# Autodesk Inventor assembly: MK3-Swerve-Module-Falcons-&-Neos
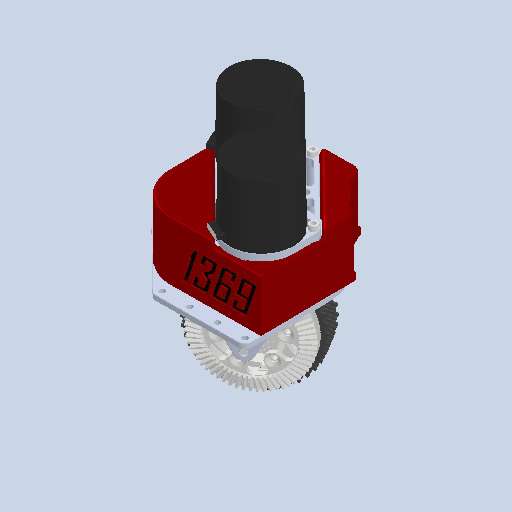
[picture p0: Inventor's stored thumbnail of the model, 512x512]
Saved by Autodesk Inventor 2024 (Build 280153000, 153)
## iProperties
Created: 2024-01-06
Part Number: MK3-Swerve-Module-Falcons-&-Neos
Document SubType Name: Assembly
Designer: rohan
Author: rohan
## Documents named in this file (27)
- C:\Users\5652160\OneDrive - Hillsborough County Public Schools\Robotics\FIRST-Robotics-Competition\Crescendo\Minotaur-Crescendo-Robot\Motion\Swerve-Modules\MK3-Swerve-Module-Neos.iam
- C:\Users\5652160\OneDrive - Hillsborough County Public Schools\Robotics\FIRST-Robotics-Competition\Crescendo\Minotaur-Crescendo-Robot\Motion\Swerve-Modules\SDS MK3 Swerve Module, Falcons, HG\MK3 Plates(Both Plates With Chamfers.ipt
- C:\Users\5652160\OneDrive - Hillsborough County Public Schools\Robotics\FIRST-Robotics-Competition\Crescendo\Minotaur-Crescendo-Robot\Electronics\NEO-Brushless-Motor.ipt
- C:\Users\5652160\OneDrive - Hillsborough County Public Schools\Robotics\FIRST-Robotics-Competition\Crescendo\Minotaur-Crescendo-Robot\Motion\Swerve-Modules\SDS MK3 Swerve Module, Falcons, HG\Spacer, #10 X 1.875, .3125 OD, 92510.ipt
- C:\Users\5652160\OneDrive - Hillsborough County Public Schools\Robotics\FIRST-Robotics-Competition\Crescendo\Minotaur-Crescendo-Robot\Motion\Swerve-Modules\SDS MK3 Swerve Module, Falcons, HG\Screw, 10-32 X 2.5, 91251A355-1.ipt
- C:\Users\5652160\OneDrive - Hillsborough County Public Schools\Robotics\FIRST-Robotics-Competition\Crescendo\Minotaur-Crescendo-Robot\Motion\Swerve-Modules\SDS MK3 Swerve Module, Falcons, HG\Screw, 10-32 X .375, 91251A340-1.ipt
- C:\Users\5652160\OneDrive - Hillsborough County Public Schools\Robotics\FIRST-Robotics-Competition\Crescendo\Minotaur-Crescendo-Robot\Motion\Swerve-Modules\SDS MK3 Swerve Module, Falcons, HG\Gear, 20DP, 16T, Falcon Spline, am-4.ipt
- C:\Users\5652160\OneDrive - Hillsborough County Public Schools\Robotics\FIRST-Robotics-Competition\Crescendo\Minotaur-Crescendo-Robot\Motion\Swerve-Modules\SDS MK3 Swerve Module, Falcons, HG\Double Gear, 20DP, 28T, 48T.ipt
- C:\Users\5652160\OneDrive - Hillsborough County Public Schools\Robotics\FIRST-Robotics-Competition\Crescendo\Minotaur-Crescendo-Robot\Motion\Swerve-Modules\SDS MK3 Swerve Module, Falcons, HG\Bearing, 6802-1.ipt
- C:\Users\5652160\OneDrive - Hillsborough County Public Schools\Robotics\FIRST-Robotics-Competition\Crescendo\Minotaur-Crescendo-Robot\Motion\Swerve-Modules\SDS MK3 Swerve Module, Falcons, HG\MK3 Center Column-1.ipt
- C:\Users\5652160\OneDrive - Hillsborough County Public Schools\Robotics\FIRST-Robotics-Competition\Crescendo\Minotaur-Crescendo-Robot\Motion\Swerve-Modules\SDS MK3 Swerve Module, Falcons, HG\Bearing, A035XPO_SA035XPO-1.ipt
- C:\Users\5652160\OneDrive - Hillsborough County Public Schools\Robotics\FIRST-Robotics-Competition\Crescendo\Minotaur-Crescendo-Robot\Motion\Swerve-Modules\SDS MK3 Swerve Module, Falcons, HG\MK3 Base Pulley-1.ipt
- C:\Users\5652160\OneDrive - Hillsborough County Public Schools\Robotics\FIRST-Robotics-Competition\Crescendo\Minotaur-Crescendo-Robot\Motion\Swerve-Modules\SDS MK3 Swerve Module, Falcons, HG\SDS 4in Wheel Assembly-1.iam
- C:\Users\5652160\OneDrive - Hillsborough County Public Schools\Robotics\FIRST-Robotics-Competition\Crescendo\Minotaur-Crescendo-Robot\Motion\Swerve-Modules\SDS MK3 Swerve Module, Falcons, HG\Gear, Bevel, KSB1.5-6015, VersaHub, .ipt
- C:\Users\5652160\OneDrive - Hillsborough County Public Schools\Robotics\FIRST-Robotics-Competition\Crescendo\Minotaur-Crescendo-Robot\Motion\Swerve-Modules\SDS MK3 Swerve Module, Falcons, HG\Bearing, am-0573, 217-2732-1.ipt
- C:\Users\5652160\OneDrive - Hillsborough County Public Schools\Robotics\FIRST-Robotics-Competition\Crescendo\Minotaur-Crescendo-Robot\Motion\Swerve-Modules\SDS MK3 Swerve Module, Falcons, HG\Wheel Mount A(Default)-1.ipt
- C:\Users\5652160\OneDrive - Hillsborough County Public Schools\Robotics\FIRST-Robotics-Competition\Crescendo\Minotaur-Crescendo-Robot\Motion\Swerve-Modules\SDS MK3 Swerve Module, Falcons, HG\Screw, Shoulder, .375 X 2.5, 5_16-18.ipt
- C:\Users\5652160\OneDrive - Hillsborough County Public Schools\Robotics\FIRST-Robotics-Competition\Crescendo\Minotaur-Crescendo-Robot\Motion\Swerve-Modules\SDS MK3 Swerve Module, Falcons, HG\MK1 Wheel Spacer-1.ipt
- C:\Users\5652160\OneDrive - Hillsborough County Public Schools\Robotics\FIRST-Robotics-Competition\Crescendo\Minotaur-Crescendo-Robot\Motion\Swerve-Modules\SDS MK3 Swerve Module, Falcons, HG\Bearing, FR8, am-0030, 217-3875-1.ipt
- C:\Users\5652160\OneDrive - Hillsborough County Public Schools\Robotics\FIRST-Robotics-Competition\Crescendo\Minotaur-Crescendo-Robot\Motion\Swerve-Modules\SDS MK3 Swerve Module, Falcons, HG\Wheel Mount B(Default)-1.ipt
- C:\Users\5652160\OneDrive - Hillsborough County Public Schools\Robotics\FIRST-Robotics-Competition\Crescendo\Minotaur-Crescendo-Robot\Motion\Swerve-Modules\SDS MK3 Swerve Module, Falcons, HG\Screw, .25-20 X 1 Socket, 91251A542-.ipt
- C:\Users\5652160\OneDrive - Hillsborough County Public Schools\Robotics\FIRST-Robotics-Competition\Crescendo\Minotaur-Crescendo-Robot\Motion\Swerve-Modules\SDS MK3 Swerve Module, Falcons, HG\Bearing, F689-ZZ-1.ipt
- C:\Users\5652160\OneDrive - Hillsborough County Public Schools\Robotics\FIRST-Robotics-Competition\Crescendo\Minotaur-Crescendo-Robot\Motion\Swerve-Modules\SDS MK3 Swerve Module, Falcons, HG\Gear, 32DP, 32T, .375 Hex Bore-1.ipt
- C:\Users\5652160\OneDrive - Hillsborough County Public Schools\Robotics\FIRST-Robotics-Competition\Crescendo\Minotaur-Crescendo-Robot\Motion\Swerve-Modules\SDS MK3 Swerve Module, Falcons, HG\MK2 Steering Shaft V3 Assembly-1.iam
- C:\Users\5652160\OneDrive - Hillsborough County Public Schools\Robotics\FIRST-Robotics-Competition\Crescendo\Minotaur-Crescendo-Robot\Motion\Swerve-Modules\SDS MK3 Swerve Module, Falcons, HG\Belt, 320-5M-09-1.ipt
- C:\Users\5652160\OneDrive - Hillsborough County Public Schools\Robotics\FIRST-Robotics-Competition\Crescendo\Minotaur-Crescendo-Robot\Structure\3D-Printed-Components\MK3-Swerve-Guard.ipt
- C:\Users\5652160\OneDrive - Hillsborough County Public Schools\Robotics\FIRST-Robotics-Competition\Crescendo\Minotaur-Crescendo-Robot\Electronics\CANcoder-Assembled.iam
## Components (37 placed, 26 different names)
1. MK3 Plates(Both Plates With Chamfers:1 — Mate:4, Mate:5, Mate:6, Mate:7, Mate:8, Mate:9, Mate:10, Mate:11, Mate:12, Mate:13, Mate:14, Mate:15, Mate:16, Mate:19, Mate:20, Mate:23, Mate:24, Mate:39, Mate:42, Mate:49, Mate:50, Mate:77, Mate:78, Mate:87, Mate:91, Mate:93, Mate:96, Mate:99, Mate:100
2. NEO-Brushless-Motor:1 — Mate:4, Mate:5, Mate:6, Mate:25
3. Spacer, #10 X 1.875, .3125 OD, 92510:1 — Mate:10, Mate:12, Mate:18
4. Spacer, #10 X 1.875, .3125 OD, 92510:2 — Mate:9, Mate:14, Mate:22, Mate:95
5. Spacer, #10 X 1.875, .3125 OD, 92510:3 — Mate:8, Mate:13, Mate:17
6. Spacer, #10 X 1.875, .3125 OD, 92510:4 — Mate:7, Mate:11, Mate:21, Mate:94
7. Screw, 10-32 X 2.5, 91251A355-1:1 — Mate:20, Mate:22
8. Screw, 10-32 X 2.5, 91251A355-1:2 — Mate:19, Mate:21, Mate:97
9. Screw, 10-32 X 2.5, 91251A355-1:3 — Mate:16, Mate:17
10. Screw, 10-32 X 2.5, 91251A355-1:4 — Mate:15, Mate:18
11. Screw, 10-32 X .375, 91251A340-1:1 — Mate:23, Mate:91, Mate:98
12. Screw, 10-32 X .375, 91251A340-1:2 — Mate:24, Mate:25
13. Gear, 20DP, 16T, Falcon Spline, am-4:1 — Mate:92
14. Double Gear, 20DP, 28T, 48T:1 — Mate:35, Mate:36, Mate:37, Mate:38, Mate:47, Mate:48
15. Bearing, 6802-1:1 — Mate:35, Mate:36
16. Bearing, 6802-1:2 — Mate:37, Mate:38
17. MK3 Center Column-1:1 — Mate:39, Mate:40, Mate:41, Mate:42, Mate:47, Mate:48, Mate:51, Mate:52, Mate:53, Mate:54
18. Bearing, 6802-1:3 — Mate:40, Mate:41
19. Bearing, A035XPO_SA035XPO-1:1 — Mate:49, Mate:50
20. MK3 Base Pulley-1:1 — Mate:51, Mate:52, Mate:53, Mate:54, Mate:70, Mate:71, Mate:72, Mate:84
21. SDS 4in Wheel Assembly-1:1 [sub-assembly] — Mate:55, Mate:56, Mate:57, Mate:58, Mate:59, Mate:64, Mate:65
22. Gear, Bevel, KSB1.5-6015, VersaHub, :1 — Mate:55, Mate:56, Mate:57
23. Bearing, am-0573, 217-2732-1:1 — Mate:58, Mate:59, Mate:60, Mate:61
24. Wheel Mount A(Default)-1:1 — Mate:60, Mate:61, Mate:62, Mate:63, Mate:70, Mate:73, Mate:74, Mate:75, Mate:76
25. Screw, Shoulder, .375 X 2.5, 5_16-18:1 — Mate:62, Mate:63, Mate:67, Mate:69
26. MK1 Wheel Spacer-1:1 — Mate:66, Mate:67, Mate:68
27. Bearing, FR8, am-0030, 217-3875-1:1 — Mate:64, Mate:65, Mate:66
28. Wheel Mount B(Default)-1:1 — Mate:68, Mate:69, Mate:71, Mate:72
29. Screw, .25-20 X 1 Socket, 91251A542-:2 — Mate:74, Mate:75
30. Screw, .25-20 X 1 Socket, 91251A542-:4 — Mate:73, Mate:76
31. Bearing, F689-ZZ-1:1 — Mate:77, Mate:78, Mate:82, Mate:83
32. Gear, 32DP, 32T, .375 Hex Bore-1:1 — Mate:79, Mate:80, Mate:81, Mate:83
33. MK2 Steering Shaft V3 Assembly-1:1 [sub-assembly] — Mate:79, Mate:80, Mate:81, Mate:82, Mate:85, Mate:86
34. Belt, 320-5M-09-1:1 — Mate:84, Mate:85, Mate:86
35. NEO-Brushless-Motor:2 — Mate:87, Mate:92, Mate:97, Mate:98
36. MK3-Swerve-Guard:1 — Mate:93, Mate:94, Mate:95
37. CANcoder-Assembled:1 [sub-assembly] — Mate:96, Mate:99, Mate:100
## Relationships (81: Mate 81)
- Mate:4: MK3 Plates(Both Plates With Chamfers:1 ↔ NEO-Brushless-Motor:1
- Mate:5: MK3 Plates(Both Plates With Chamfers:1 ↔ NEO-Brushless-Motor:1
- Mate:6: MK3 Plates(Both Plates With Chamfers:1 ↔ NEO-Brushless-Motor:1
- Mate:7: MK3 Plates(Both Plates With Chamfers:1 ↔ Spacer, #10 X 1.875, .3125 OD, 92510:4
- Mate:8: MK3 Plates(Both Plates With Chamfers:1 ↔ Spacer, #10 X 1.875, .3125 OD, 92510:3
- Mate:9: MK3 Plates(Both Plates With Chamfers:1 ↔ Spacer, #10 X 1.875, .3125 OD, 92510:2
- Mate:10: MK3 Plates(Both Plates With Chamfers:1 ↔ Spacer, #10 X 1.875, .3125 OD, 92510:1
- Mate:11: MK3 Plates(Both Plates With Chamfers:1 ↔ Spacer, #10 X 1.875, .3125 OD, 92510:4
- Mate:12: MK3 Plates(Both Plates With Chamfers:1 ↔ Spacer, #10 X 1.875, .3125 OD, 92510:1
- Mate:13: MK3 Plates(Both Plates With Chamfers:1 ↔ Spacer, #10 X 1.875, .3125 OD, 92510:3
- Mate:14: MK3 Plates(Both Plates With Chamfers:1 ↔ Spacer, #10 X 1.875, .3125 OD, 92510:2
- Mate:15: MK3 Plates(Both Plates With Chamfers:1 ↔ Screw, 10-32 X 2.5, 91251A355-1:4
- Mate:16: MK3 Plates(Both Plates With Chamfers:1 ↔ Screw, 10-32 X 2.5, 91251A355-1:3
- Mate:17: Spacer, #10 X 1.875, .3125 OD, 92510:3 ↔ Screw, 10-32 X 2.5, 91251A355-1:3
- Mate:18: Spacer, #10 X 1.875, .3125 OD, 92510:1 ↔ Screw, 10-32 X 2.5, 91251A355-1:4
- Mate:19: MK3 Plates(Both Plates With Chamfers:1 ↔ Screw, 10-32 X 2.5, 91251A355-1:2
- Mate:20: MK3 Plates(Both Plates With Chamfers:1 ↔ Screw, 10-32 X 2.5, 91251A355-1:1
- Mate:21: Spacer, #10 X 1.875, .3125 OD, 92510:4 ↔ Screw, 10-32 X 2.5, 91251A355-1:2
- Mate:22: Spacer, #10 X 1.875, .3125 OD, 92510:2 ↔ Screw, 10-32 X 2.5, 91251A355-1:1
- Mate:23: MK3 Plates(Both Plates With Chamfers:1 ↔ Screw, 10-32 X .375, 91251A340-1:1
- Mate:24: MK3 Plates(Both Plates With Chamfers:1 ↔ Screw, 10-32 X .375, 91251A340-1:2
- Mate:25: NEO-Brushless-Motor:1 ↔ Screw, 10-32 X .375, 91251A340-1:2
- Mate:35: Double Gear, 20DP, 28T, 48T:1 ↔ Bearing, 6802-1:1
- Mate:36: Double Gear, 20DP, 28T, 48T:1 ↔ Bearing, 6802-1:1
- Mate:37: Double Gear, 20DP, 28T, 48T:1 ↔ Bearing, 6802-1:2
- Mate:38: Double Gear, 20DP, 28T, 48T:1 ↔ Bearing, 6802-1:2
- Mate:39: MK3 Plates(Both Plates With Chamfers:1 ↔ MK3 Center Column-1:1
- Mate:40: MK3 Center Column-1:1 ↔ Bearing, 6802-1:3
- Mate:41: MK3 Center Column-1:1 ↔ Bearing, 6802-1:3
- Mate:42: MK3 Plates(Both Plates With Chamfers:1 ↔ MK3 Center Column-1:1
- Mate:47: Double Gear, 20DP, 28T, 48T:1 ↔ MK3 Center Column-1:1
- Mate:48: Double Gear, 20DP, 28T, 48T:1 ↔ MK3 Center Column-1:1
- Mate:49: MK3 Plates(Both Plates With Chamfers:1 ↔ Bearing, A035XPO_SA035XPO-1:1
- Mate:50: MK3 Plates(Both Plates With Chamfers:1 ↔ Bearing, A035XPO_SA035XPO-1:1
- Mate:51: MK3 Center Column-1:1 ↔ MK3 Base Pulley-1:1
- Mate:52: MK3 Center Column-1:1 ↔ MK3 Base Pulley-1:1
- Mate:53: MK3 Center Column-1:1 ↔ MK3 Base Pulley-1:1
- Mate:54: MK3 Center Column-1:1 ↔ MK3 Base Pulley-1:1
- Mate:55: SDS 4in Wheel Assembly-1:1 ↔ Gear, Bevel, KSB1.5-6015, VersaHub, :1
- Mate:56: SDS 4in Wheel Assembly-1:1 ↔ Gear, Bevel, KSB1.5-6015, VersaHub, :1
- Mate:57: SDS 4in Wheel Assembly-1:1 ↔ Gear, Bevel, KSB1.5-6015, VersaHub, :1
- Mate:58: SDS 4in Wheel Assembly-1:1 ↔ Bearing, am-0573, 217-2732-1:1
- Mate:59: SDS 4in Wheel Assembly-1:1 ↔ Bearing, am-0573, 217-2732-1:1
- Mate:60: Bearing, am-0573, 217-2732-1:1 ↔ Wheel Mount A(Default)-1:1
- Mate:61: Bearing, am-0573, 217-2732-1:1 ↔ Wheel Mount A(Default)-1:1
- Mate:62: Wheel Mount A(Default)-1:1 ↔ Screw, Shoulder, .375 X 2.5, 5_16-18:1
- Mate:63: Wheel Mount A(Default)-1:1 ↔ Screw, Shoulder, .375 X 2.5, 5_16-18:1
- Mate:64: SDS 4in Wheel Assembly-1:1 ↔ Bearing, FR8, am-0030, 217-3875-1:1
- Mate:65: SDS 4in Wheel Assembly-1:1 ↔ Bearing, FR8, am-0030, 217-3875-1:1
- Mate:66: MK1 Wheel Spacer-1:1 ↔ Bearing, FR8, am-0030, 217-3875-1:1
- Mate:67: Screw, Shoulder, .375 X 2.5, 5_16-18:1 ↔ MK1 Wheel Spacer-1:1
- Mate:68: MK1 Wheel Spacer-1:1 ↔ Wheel Mount B(Default)-1:1
- Mate:69: Screw, Shoulder, .375 X 2.5, 5_16-18:1 ↔ Wheel Mount B(Default)-1:1
- Mate:70: MK3 Base Pulley-1:1 ↔ Wheel Mount A(Default)-1:1
- Mate:71: MK3 Base Pulley-1:1 ↔ Wheel Mount B(Default)-1:1
- Mate:72: MK3 Base Pulley-1:1 ↔ Wheel Mount B(Default)-1:1
- Mate:73: Wheel Mount A(Default)-1:1 ↔ Screw, .25-20 X 1 Socket, 91251A542-:4
- Mate:74: Wheel Mount A(Default)-1:1 ↔ Screw, .25-20 X 1 Socket, 91251A542-:2
- Mate:75: Wheel Mount A(Default)-1:1 ↔ Screw, .25-20 X 1 Socket, 91251A542-:2
- Mate:76: Wheel Mount A(Default)-1:1 ↔ Screw, .25-20 X 1 Socket, 91251A542-:4
- Mate:77: MK3 Plates(Both Plates With Chamfers:1 ↔ Bearing, F689-ZZ-1:1
- Mate:78: MK3 Plates(Both Plates With Chamfers:1 ↔ Bearing, F689-ZZ-1:1
- Mate:79: Gear, 32DP, 32T, .375 Hex Bore-1:1 ↔ MK2 Steering Shaft V3 Assembly-1:1
- Mate:80: Gear, 32DP, 32T, .375 Hex Bore-1:1 ↔ MK2 Steering Shaft V3 Assembly-1:1
- Mate:81: Gear, 32DP, 32T, .375 Hex Bore-1:1 ↔ MK2 Steering Shaft V3 Assembly-1:1
- Mate:82: Bearing, F689-ZZ-1:1 ↔ MK2 Steering Shaft V3 Assembly-1:1
- Mate:83: Bearing, F689-ZZ-1:1 ↔ Gear, 32DP, 32T, .375 Hex Bore-1:1
- Mate:84: MK3 Base Pulley-1:1 ↔ Belt, 320-5M-09-1:1
- Mate:85: MK2 Steering Shaft V3 Assembly-1:1 ↔ Belt, 320-5M-09-1:1
- Mate:86 (0.2032 mm): MK2 Steering Shaft V3 Assembly-1:1 ↔ Belt, 320-5M-09-1:1
- Mate:87: MK3 Plates(Both Plates With Chamfers:1 ↔ NEO-Brushless-Motor:2
- Mate:91: MK3 Plates(Both Plates With Chamfers:1 ↔ Screw, 10-32 X .375, 91251A340-1:1
- Mate:92: Gear, 20DP, 16T, Falcon Spline, am-4:1 ↔ NEO-Brushless-Motor:2
- Mate:93: MK3 Plates(Both Plates With Chamfers:1 ↔ MK3-Swerve-Guard:1
- Mate:94: Spacer, #10 X 1.875, .3125 OD, 92510:4 ↔ MK3-Swerve-Guard:1
- Mate:95: Spacer, #10 X 1.875, .3125 OD, 92510:2 ↔ MK3-Swerve-Guard:1
- Mate:96: MK3 Plates(Both Plates With Chamfers:1 ↔ CANcoder-Assembled:1
- Mate:97: Screw, 10-32 X 2.5, 91251A355-1:2 ↔ NEO-Brushless-Motor:2
- Mate:98: Screw, 10-32 X .375, 91251A340-1:1 ↔ NEO-Brushless-Motor:2
- Mate:99: MK3 Plates(Both Plates With Chamfers:1 ↔ CANcoder-Assembled:1
- Mate:100: MK3 Plates(Both Plates With Chamfers:1 ↔ CANcoder-Assembled:1
